# Autodesk Inventor assembly: RollerAssemblyBearing
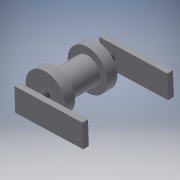
[picture p0: Inventor's stored thumbnail of the model, 180x180]
Saved by Autodesk Inventor 2018.3 (Build 223284000, 284)
## iProperties
Created: 2020-01-25
Part Number: RollerAssemblyBearing
Document SubType Name: Assembly
Designer: 22jungchan
Mass: 9.41301 g
Surface Area: 68.0408 cm^2
Volume: 9.41301 cm^3
Density: 1 g/cm^3
Author: 22jungchan
## Documents named in this file (5)
- C:\Users\22perngrac\Documents\GrabCAD\Infinite Recharge 2020\Build season\CLB_024_RollerAssembly(Bearing)S3.iam
- C:\Users\22perngrac\Documents\GrabCAD\Infinite Recharge 2020\Build season\CLB_015_RollerShaftS3.ipt
- C:\Users\22perngrac\Documents\GrabCAD\Infinite Recharge 2020\Build season\CLB_010_RollerSquareBracket.ipt
- C:\Users\22perngrac\Documents\GrabCAD\Infinite Recharge 2020\Build season\CLB_012_RollerSpacer2(Bearing)-S3.ipt
- C:\Users\22perngrac\Documents\GrabCAD\Infinite Recharge 2020\Build season\CLB_014_Bearing.ipt
## Components (6 placed, 4 different names)
1. CLB_015_RollerShaftS3:1 — Insert:1, Insert:4
2. CLB_010_RollerSquareBracket:3 — Insert:1, Angle:1
3. CLB_010_RollerSquareBracket:4 — Insert:4, Angle:1, Insert:7
4. CLB_012_RollerSpacer2(Bearing)-S3:1 — Mate:1, Insert:5, Insert:6, Insert:7
5. CLB_014_Bearing:3 — Insert:5
6. CLB_014_Bearing:4 — Mate:1, Insert:6
## Relationships (7: Insert 5, Mate 1, Angle 1)
- Insert:1: CLB_015_RollerShaftS3:1 ↔ CLB_010_RollerSquareBracket:3
- Insert:4: CLB_015_RollerShaftS3:1 ↔ CLB_010_RollerSquareBracket:4
- Mate:1: CLB_012_RollerSpacer2(Bearing)-S3:1 ↔ CLB_014_Bearing:4
- Angle:1 (0 deg): CLB_010_RollerSquareBracket:3 ↔ CLB_010_RollerSquareBracket:4
- Insert:5: CLB_012_RollerSpacer2(Bearing)-S3:1 ↔ CLB_014_Bearing:3
- Insert:6: CLB_012_RollerSpacer2(Bearing)-S3:1 ↔ CLB_014_Bearing:4
- Insert:7 (7.62 mm): CLB_010_RollerSquareBracket:4 ↔ CLB_012_RollerSpacer2(Bearing)-S3:1
